# Autodesk Inventor assembly: 5-15
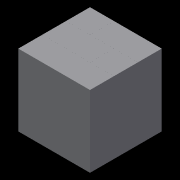
[picture p0: Inventor's stored thumbnail of the model, 180x180]
Saved by Autodesk Inventor 2017 (Build 210142000, 142)
## iProperties
Part Number: 5-15
Material: 一般
Document SubType Name: Assembly
Designer: r0909
Author: r0909
## Documents named in this file (5)
- C:\Users\r0909\Desktop\inventor\5-15.iam
- C:\Users\r0909\Desktop\inventor\5-11.ipt
- C:\Users\r0909\Desktop\inventor\5-12.ipt
- C:\Users\r0909\Desktop\inventor\5-13.ipt
- C:\Users\r0909\Desktop\inventor\5-14.ipt
## Components (7 placed, 4 different names)
1. 5-11:1 — 貼合:12, 貼合:13, 貼合:14
2. 5-12:1 — 貼合:9, 貼合:10, 貼合:11, 貼合:13
3. 5-13:1 — 貼合:1, 齊平:1, 齊平:2, 齊平:3, 貼合:2, 齊平:4, 齊平:5, 貼合:4, 貼合:5, 齊平:6, 齊平:7, 貼合:8
4. 5-14:1 — 齊平:5, 貼合:3, 貼合:4, 貼合:6, 貼合:7, 貼合:10, 貼合:11
5. 5-13:2 — 齊平:3, 貼合:2, 齊平:4, 貼合:3
6. 5-13:3 — 貼合:5, 貼合:6, 齊平:6, 貼合:9
7. 5-13:4 — 貼合:7, 齊平:7, 貼合:8, 貼合:12, 貼合:14
## Relationships (21: Mate 14, Flush 7)
- 貼合:1 [Mate]: 5-13:1
- 齊平:1 [Flush]: 5-13:1
- 齊平:2 [Flush]: 5-13:1
- 齊平:3 [Flush]: 5-13:1 ↔ 5-13:2
- 貼合:2 [Mate]: 5-13:1 ↔ 5-13:2
- 齊平:4 [Flush]: 5-13:1 ↔ 5-13:2
- 齊平:5 [Flush]: 5-13:1 ↔ 5-14:1
- 貼合:3 [Mate]: 5-14:1 ↔ 5-13:2
- 貼合:4 [Mate]: 5-13:1 ↔ 5-14:1
- 貼合:5 [Mate]: 5-13:1 ↔ 5-13:3
- 貼合:6 [Mate]: 5-14:1 ↔ 5-13:3
- 齊平:6 [Flush]: 5-13:1 ↔ 5-13:3
- 貼合:7 [Mate]: 5-14:1 ↔ 5-13:4
- 齊平:7 [Flush]: 5-13:1 ↔ 5-13:4
- 貼合:8 [Mate]: 5-13:1 ↔ 5-13:4
- 貼合:9 [Mate]: 5-12:1 ↔ 5-13:3
- 貼合:10 [Mate]: 5-12:1 ↔ 5-14:1
- 貼合:11 [Mate]: 5-12:1 ↔ 5-14:1
- 貼合:12 [Mate]: 5-11:1 ↔ 5-13:4
- 貼合:13 [Mate]: 5-11:1 ↔ 5-12:1
- 貼合:14 [Mate]: 5-11:1 ↔ 5-13:4
